# Autodesk Inventor assembly: !Drivebay Left
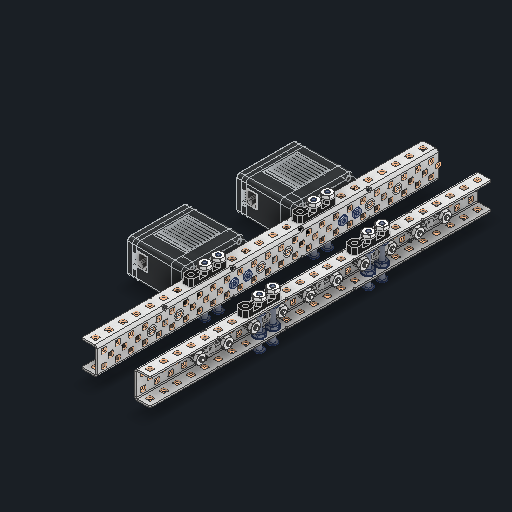
[picture p0: Inventor's stored thumbnail of the model, 512x512]
Saved by Autodesk Inventor 2025.1 (Build 291241000, 241)
## iProperties
Created: 2024-11-28
Part Number: !Drivebay Left
Document SubType Name: Assembly
Designer: avere
Author: avere
## Documents named in this file (3)
- C:\Users\avere\VEX\High Stakes\CAD\Codie\Chassis\Drivebay Left\!Drivebay Left.iam
- C:\Users\avere\VEX\High Stakes\CAD\Codie\Chassis\Drivebay Left\Outer.iam
- C:\Users\avere\VEX\High Stakes\CAD\Codie\Chassis\Drivebay Left\Inner\Inner.iam
## Components (2 placed, 2 different names)
1. Outer:1 [sub-assembly] — Mate:1, Mate:2, Flush:1
2. Inner:1 [sub-assembly] — Flush:2, Mate:3, Flush:3
## Relationships (6: Mate 3, Flush 3)
- Mate:1 (17.4625 mm): Outer:1
- Mate:2 (41.275 mm): Outer:1
- Flush:1 (-158.75 mm): Outer:1
- Flush:2 (-158.75 mm): Inner:1
- Mate:3 (41.275 mm): Inner:1
- Flush:3 (17.4625 mm): Inner:1
